# Autodesk Inventor assembly: Assembly esp32
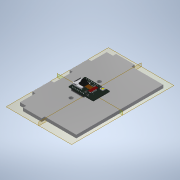
[picture p0: Inventor's stored thumbnail of the model, 180x180]
Saved by Autodesk Inventor 2021 (Build 250183000, 183)
## iProperties
Manager: Pierloot J.
Company: Emmaüs Bovenbouw Aalter
Created: 2021-01-30
Part Number: Assembly esp32
Catalog Web Link: http://emmausbovenbouw.op-weg.be/
Vendor: Emmaüs Bovenbouw Aalter
Document SubType Name: Assembly
Designer: Antho
Engineer: Declercq St.
Authority: Declercq St.
Title: Algemene Projecttitel
Author: Antho
## Documents named in this file (3)
- F:\GIP 6EM\Assembly\Assembly esp32.iam
- F:\GIP 6EM\Frame\Plaat voor.ipt
- F:\GIP 6EM\Bevestigingen\ESP3-CAM v5 - black pcb.iam
## Components (2 placed, 2 different names)
1. Plaat voor:1 — Mate:1, Mate:2, Mate:3
2. ESP3-CAM v5 - black pcb:1 [sub-assembly] — Mate:1, Mate:2, Mate:3
## Relationships (3: Mate 3)
- Mate:1: Plaat voor:1 ↔ ESP3-CAM v5 - black pcb:1
- Mate:2: Plaat voor:1 ↔ ESP3-CAM v5 - black pcb:1
- Mate:3: Plaat voor:1 ↔ ESP3-CAM v5 - black pcb:1
